# Autodesk Inventor assembly: Flashlight
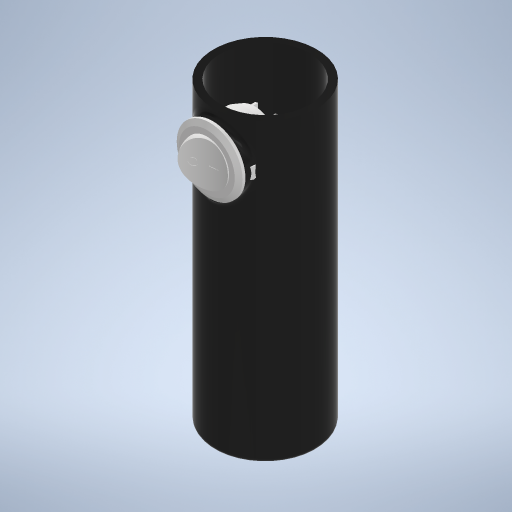
[picture p0: Inventor's stored thumbnail of the model, 512x512]
Saved by Autodesk Inventor 2024.2 (Build 282272000, 272)
## iProperties
Created: 2025-04-09
Part Number: Flashlight
Document SubType Name: Assembly
Designer: Svend
Author: Svend
## Documents named in this file (4)
- C:\Semesterprojekt\semesterproject_4_6\Inventor\Flashlight.iam
- C:\Semesterprojekt\semesterproject_4_6\Inventor\Flash_light.ipt
- C:\Users\Svend\OneDrive - Syddansk Universitet\2 semester\Semesterprojekt i autonome robotter\HG37-300-AB-00\3D\Battery_Holder_3AA_V1.ipt
- C:\Semesterprojekt\semesterproject_4_6\Inventor\161130345-9-xb-rs601c-1020011bb-zp\xb-rs601c-1020011bb-zp.iam
## Components (3 placed, 3 different names)
1. Flash_light:1 — Mate:1, Mate:2, Mate:3, Mate:4
2. Battery_Holder_3AA_V1:1 — Mate:1, Mate:2
3. xb-rs601c-1020011bb-zp:1 [sub-assembly] — Mate:3, Mate:4
## Relationships (4: Mate 4)
- Mate:1: Flash_light:1 ↔ Battery_Holder_3AA_V1:1
- Mate:2: Flash_light:1 ↔ Battery_Holder_3AA_V1:1
- Mate:3: Flash_light:1 ↔ xb-rs601c-1020011bb-zp:1
- Mate:4: Flash_light:1 ↔ xb-rs601c-1020011bb-zp:1
